# Autodesk Inventor assembly: dtmotorgears
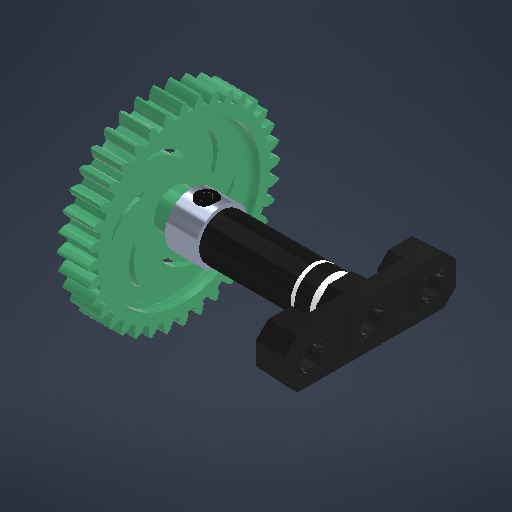
[picture p0: Inventor's stored thumbnail of the model, 512x512]
Saved by Autodesk Inventor 2026.1 (Build 301233000, 233)
## iProperties
Created: 2025-08-03
Part Number: dtmotorgears
Document SubType Name: Assembly
Designer: roejo
Author: roejo
## Documents named in this file (11)
- C:\Users\roejo\OneDrive\Documents\3284b-cad-2025\Robots\Highlander\SubAssemblies\dtmotorgears.iam
- C:\Users\roejo\OneDrive\Documents\3284b-cad-2025\Library\VEX-CAD-Inventor-1.4.2\Motion\Gears\LS 36T Gear.ipt
- C:\Users\roejo\OneDrive\Documents\3284b-cad-2025\Library\VEX-CAD-Inventor-1.4.2\Motion\Spacers\Washer Teflon\TWasher .375 OD x .06250.ipt
- C:\Users\roejo\OneDrive\Documents\3284b-cad-2025\Library\VEX-CAD-Inventor-1.4.2\Motion\Spacers\Washer Teflon.ipt
- C:\Users\roejo\OneDrive\Documents\3284b-cad-2025\Library\VEX-CAD-Inventor-1.4.2\Motion\Shaft LS\Shaft Collar Metal\Shaft Collar Set Screw.ipt
- C:\Users\roejo\OneDrive\Documents\3284b-cad-2025\Library\VEX-CAD-Inventor-1.4.2\Motion\Spacers\Spacer Nylon .375 OD\NSpacer .375 OD x .500.ipt
- C:\Users\roejo\OneDrive\Documents\3284b-cad-2025\Library\VEX-CAD-Inventor-1.4.2\Motion\Spacers\Spacer Nylon .375 OD.ipt
- C:\Users\roejo\OneDrive\Documents\3284b-cad-2025\Library\VEX-CAD-Inventor-1.4.2\Motion\Spacers\Spacer Nylon .375 OD\NSpacer .375 OD x .125.ipt
- C:\Users\roejo\OneDrive\Documents\3284b-cad-2025\Library\VEX-CAD-Inventor-1.4.2\Motion\Spacers\Washer Teflon\TWasher .375 OD x .03125.ipt
- C:\Users\roejo\OneDrive\Documents\3284b-cad-2025\Library\VEX-CAD-Inventor-1.4.2\Motion\Spacers\Spacer Nylon .375 OD\NSpacer .375 OD x .250.ipt
- C:\Users\roejo\OneDrive\Documents\3284b-cad-2025\Library\VEX-CAD-Inventor-1.4.2\Motion\Shaft LS\Bearing Flat.ipt
## Components (9 placed, 8 different names)
1. LS 36T Gear:1 — Insert:1, Insert:2
2. TWasher .375 OD x .06250:1 — Insert:1
3. Shaft Collar Set Screw:1 — Insert:2, Insert:3
4. NSpacer .375 OD x .500:1 — Insert:3, Insert:8
5. NSpacer .375 OD x .125:3 — Insert:6, Insert:7
6. TWasher .375 OD x .06250:2 — Insert:7, Insert:10
7. TWasher .375 OD x .03125:3 — Insert:6, Insert:9
8. NSpacer .375 OD x .250:4 — Insert:8, Insert:9
9. Bearing Flat:1 — Insert:10
## Relationships (8: Insert 8)
- Insert:1: LS 36T Gear:1 ↔ TWasher .375 OD x .06250:1
- Insert:2: LS 36T Gear:1 ↔ Shaft Collar Set Screw:1
- Insert:3: Shaft Collar Set Screw:1 ↔ NSpacer .375 OD x .500:1
- Insert:6: NSpacer .375 OD x .125:3 ↔ TWasher .375 OD x .03125:3
- Insert:7: NSpacer .375 OD x .125:3 ↔ TWasher .375 OD x .06250:2
- Insert:8: NSpacer .375 OD x .500:1 ↔ NSpacer .375 OD x .250:4
- Insert:9: TWasher .375 OD x .03125:3 ↔ NSpacer .375 OD x .250:4
- Insert:10: TWasher .375 OD x .06250:2 ↔ Bearing Flat:1
